# Autodesk Inventor assembly: Mecanum with supports
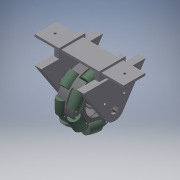
[picture p0: Inventor's stored thumbnail of the model, 180x180]
Saved by Autodesk Inventor 2018 (Build 220112000, 112)
## iProperties
Created: 2018-05-02
Part Number: Mecanum with supports
Document SubType Name: Assembly
Designer: Ajith Thomas
Author: Ajith Thomas
## Documents named in this file (8)
- C:\Users\Ajith Thomas\Dropbox\Gas_Sensing_Robot\FumeBot-Design\Mecanum with supports.iam
- C:\Users\Ajith Thomas\Dropbox\Gas_Sensing_Robot\FumeBot-Design\Mecanum\Mecanum Wheel.iam
- C:\Users\Ajith Thomas\Dropbox\Gas_Sensing_Robot\FumeBot-Design\M4 Nut.ipt
- C:\Users\Ajith Thomas\Dropbox\Gas_Sensing_Robot\FumeBot-Design\Bearing.ipt
- C:\Users\Ajith Thomas\Dropbox\Gas_Sensing_Robot\FumeBot-Design\Mecanum wheel threaded rod.ipt
- C:\Users\Ajith Thomas\Dropbox\Gas_Sensing_Robot\FumeBot-Design\Mecanum wheel support.ipt
- C:\Users\Ajith Thomas\Dropbox\Gas_Sensing_Robot\FumeBot-Design\Bearing lockers.ipt
- C:\Users\Ajith Thomas\Dropbox\Gas_Sensing_Robot\FumeBot-Design\Mechanum support lock bar.ipt
## Components (19 placed, 7 different names)
1. Mecanum Wheel:1 [sub-assembly] — Insert:1, Insert:5, Mate:1, Mate:7
2. M4 Nut:1 — Insert:1, Insert:2
3. M4 Nut:2 — Insert:2, Insert:3
4. M4 Nut:3 — Insert:3, Insert:4
5. M4 Nut:4 — Insert:4, Insert:9
6. M4 Nut:5 — Insert:5, Insert:6
7. M4 Nut:6 — Insert:6, Insert:7
8. M4 Nut:7 — Insert:7, Insert:8
9. M4 Nut:8 — Insert:8, Insert:10
10. M4 Nut:9 — Insert:11
11. M4 Nut:10 — Insert:12, Mate:2
12. Bearing:1 — Insert:9, Insert:12, Flush:1
13. Bearing:2 — Insert:10, Insert:11, Mate:3, Flush:3
14. Mecanum wheel threaded rod:1 — Mate:1, Mate:2, Mate:6
15. Mecanum wheel support:1 — Flush:1, Flush:2, Flush:4, Mate:7, Symmetry:1
16. Bearing lockers:1 — Flush:2
17. Mecanum wheel support:2 — Mate:3, Flush:3, Flush:4, Mate:4, Mate:5, Symmetry:1
18. Bearing lockers:2 — Mate:4, Mate:5, Mate:6
19. Mechanum support lock bar:1 — Flush:5
## Relationships (25: Insert 12, Mate 7, Flush 5, Symmetry 1)
- Insert:1: Mecanum Wheel:1 ↔ M4 Nut:1
- Insert:2: M4 Nut:1 ↔ M4 Nut:2
- Insert:3: M4 Nut:2 ↔ M4 Nut:3
- Insert:4: M4 Nut:3 ↔ M4 Nut:4
- Insert:5: Mecanum Wheel:1 ↔ M4 Nut:5
- Insert:6: M4 Nut:5 ↔ M4 Nut:6
- Insert:7: M4 Nut:6 ↔ M4 Nut:7
- Insert:8: M4 Nut:7 ↔ M4 Nut:8
- Insert:9: M4 Nut:4 ↔ Bearing:1
- Insert:10: M4 Nut:8 ↔ Bearing:2
- Insert:11: M4 Nut:9 ↔ Bearing:2
- Insert:12: M4 Nut:10 ↔ Bearing:1
- Mate:1: Mecanum Wheel:1 ↔ Mecanum wheel threaded rod:1
- Mate:2: M4 Nut:10 ↔ Mecanum wheel threaded rod:1
- Flush:1: Bearing:1 ↔ Mecanum wheel support:1
- Flush:2: Mecanum wheel support:1 ↔ Bearing lockers:1
- Mate:3: Bearing:2 ↔ Mecanum wheel support:2
- Flush:3: Bearing:2 ↔ Mecanum wheel support:2
- Flush:4: Mecanum wheel support:1 ↔ Mecanum wheel support:2
- Mate:4: Mecanum wheel support:2 ↔ Bearing lockers:2
- Mate:5: Mecanum wheel support:2 ↔ Bearing lockers:2
- Mate:6: Mecanum wheel threaded rod:1 ↔ Bearing lockers:2
- Mate:7: Mecanum Wheel:1 ↔ Mecanum wheel support:1
- Symmetry:1: Mecanum wheel support:1 ↔ Mecanum wheel support:2
- Flush:5: Mechanum support lock bar:1
